# Autodesk Inventor assembly: am-XXXX - 57 Sport 500 Hex Output Plug
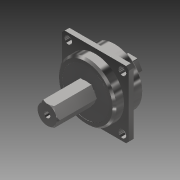
[picture p0: Inventor's stored thumbnail of the model, 180x180]
Saved by Autodesk Inventor 2018 (Build 220112000, 112)
## iProperties
Created: 2017-11-21
Part Number: am-XXXX - 57 Sport 500 Hex Output Plug
Document SubType Name: Assembly
Designer: PhillipD
Author: PhillipD
Revision Number: ANY
## Documents named in this file (5)
- D:\FIRST 2018\FIRST 2018 Inventor\FIRST 2018 Black Tote\RedLine Motor Kit\am-XXXX - 57 Sport 500 Hex Output Plug.iam
- D:\FIRST 2018\FIRST 2018 Inventor\FIRST 2018 Black Tote\RedLine Motor Kit\am-XXXX - 57 Sport 500 Hex Shaft.ipt
- D:\FIRST 2018\FIRST 2018 Inventor\FIRST 2018 Black Tote\RedLine Motor Kit\Output Block.ipt
- D:\FIRST 2018\FIRST 2018 Inventor\FIRST 2018 Black Tote\RedLine Motor Kit\FR8ZZ Bearing.ipt
- D:\FIRST 2018\FIRST 2018 Inventor\FIRST 2018 Black Tote\RedLine Motor Kit\retaining Ring 0500 - Mcm 98410A122_98410A122.ipt
## Components (5 placed, 5 different names)
1. am-XXXX - 57 Sport 500 Hex Shaft_15 — Mate:1, Mate:2
2. Output Block_16
3. FR8ZZ Bearing_17
4. FR8ZZ Bearing_18 — Mate:1, Mate:2
5. retaining Ring 0500 - Mcm 98410A122_98410A122_19
## Relationships (2: Mate 2)
- Mate:1: am-XXXX - 57 Sport 500 Hex Shaft_15 ↔ FR8ZZ Bearing_18
- Mate:2: am-XXXX - 57 Sport 500 Hex Shaft_15 ↔ FR8ZZ Bearing_18
